# Autodesk Inventor assembly: robotassembly1
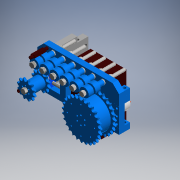
[picture p0: Inventor's stored thumbnail of the model, 180x180]
Saved by Autodesk Inventor 2016 (Build 200138000, 138)
## iProperties
Created: 2016-05-14
Part Number: robotassembly1
Document SubType Name: Assembly
Designer: hesaon
Author: hesaon
## Documents named in this file (22)
- C:\Users\hesaon\Documents\Killer-Bot-2016\AutodeskWorkspace\robotassembly1.iam
- C:\Users\hesaon\Documents\Killer-Bot-2016\AutodeskWorkspace\motorHolder57mmVer2.ipt
- C:\Users\hesaon\Documents\Killer-Bot-2016\AutodeskWorkspace\37D mm metal gearmotor.ipt
- C:\Users\hesaon\Documents\Killer-Bot-2016\AutodeskWorkspace\mountingHub6mm.ipt
- C:\Users\hesaon\Documents\Killer-Bot-2016\AutodeskWorkspace\sprocketsHolder.ipt
- C:\Users\hesaon\Documents\Killer-Bot-2016\AutodeskWorkspace\BigSprocket2.ipt
- C:\Users\hesaon\Documents\Killer-Bot-2016\AutodeskWorkspace\tracks_center.ipt
- C:\Users\hesaon\Documents\Killer-Bot-2016\AutodeskWorkspace\outerBigSprocket2.ipt
- C:\Users\hesaon\Documents\Killer-Bot-2016\AutodeskWorkspace\framesideRight.ipt
- C:\Users\hesaon\Documents\Killer-Bot-2016\AutodeskWorkspace\smallSprocketHolder.ipt
- C:\Users\hesaon\Documents\Killer-Bot-2016\AutodeskWorkspace\smallSprocket2.ipt
- C:\Users\hesaon\Documents\Killer-Bot-2016\AutodeskWorkspace\frameBack.ipt
- C:\Users\hesaon\Documents\Killer-Bot-2016\AutodeskWorkspace\pin5x60.ipt
- C:\Users\hesaon\Documents\Killer-Bot-2016\AutodeskWorkspace\smallSprocketFixture.ipt
- C:\Users\hesaon\Documents\Killer-Bot-2016\AutodeskWorkspace\roller.ipt
- C:\Users\hesaon\Documents\Killer-Bot-2016\AutodeskWorkspace\frameBottomRight.ipt
- C:\Users\hesaon\Documents\Killer-Bot-2016\AutodeskWorkspace\washer6mm.ipt
- C:\Users\hesaon\Documents\Killer-Bot-2016\AutodeskWorkspace\rollerdistance.ipt
- C:\Users\hesaon\Documents\Killer-Bot-2016\AutodeskWorkspace\nut6mm.ipt
- C:\Users\hesaon\Documents\Killer-Bot-2016\AutodeskWorkspace\bolt.ipt
- C:\Users\hesaon\Documents\Killer-Bot-2016\AutodeskWorkspace\battery.ipt
- C:\Users\hesaon\Documents\Killer-Bot-2016\AutodeskWorkspace\rollerdistanceShort.ipt
## Components (79 placed, 20 different names)
1. motorHolder57mmVer2:1 — Insert:1, Insert:2, Insert:98, Insert:99
2. 37D mm metal gearmotor:1 — Insert:1, Insert:2, Insert:3
3. mountingHub6mm:1 — Insert:3, Insert:9, Insert:10
4. sprocketsHolder:2 — Insert:7, Insert:8, Mate:1, Mate:2, Mate:3, Mate:4
5. Roller Chain Sprocket1:2 — Insert:7, Insert:8
6. Outer big sprocket:1 — Mate:1, Mate:2, Mate:3, Mate:4, Insert:9, Insert:10
7. framesideRight:1 — Flush:1, Insert:27, Insert:28, Insert:37, Flush:6, Flush:7, Insert:98, Insert:99, Insert:100, Insert:101, Mate:6, Mate:8
8. smallSprocketHolder:1 — Insert:13, Insert:14, Insert:15, Insert:16
9. Roller Chain Sprocket1:3 — Insert:13, Insert:14, Insert:93
10. Roller Chain Sprocket1:4 — Insert:15, Insert:16, Insert:17, Insert:92, Insert:94
11. tracks_center:2 — Insert:17
12. frameBack:1 — Flush:1, Flush:7, Insert:100, Insert:101
13. pin5x60:1 — Insert:27, Cylindrical:2
14. pin5x60:2 — Insert:28, Cylindrical:1
15. smallSprocketFixture:1 — Cylindrical:1, Cylindrical:2, Insert:91, Insert:95
16. roller:2 — Tangent:1, Flush:3, Flush:4, Insert:55, Insert:69, Insert:104
17. roller:3 — Insert:54, Insert:68, Insert:103, Insert:105
18. roller:4 — Insert:53, Insert:67, Insert:108
19. roller:5 — Insert:52, Insert:66, Insert:115
20. roller:6 — Insert:51, Insert:65, Insert:106
21. frameBottomRight:1 — Insert:37, Flush:6, Insert:71, Insert:72, Insert:73, Insert:74, Insert:75, Insert:76, Mate:7, Insert:103, Insert:104, Insert:105, Insert:106, Insert:107, Insert:108, Insert:115, Insert:116, Angle:1, Insert:117, Angle:2, Insert:118, Angle:3, Insert:119, Angle:4, Insert:120, Angle:5, Insert:121, Angle:6
22. tracks_center:3 — Tangent:1, Flush:3, Flush:4
23. roller:7 — Insert:50, Insert:64, Insert:107
24. washer6mm:1 — Insert:53, Insert:112
25. washer6mm:2 — Insert:51, Insert:110
26. washer6mm:3 — Insert:60
27. washer6mm:4 — Insert:59
28. washer6mm:5 — Insert:58
29. washer6mm:6 — Insert:61
30. washer6mm:7 — Insert:52, Insert:111
31. washer6mm:8 — Insert:56
32. washer6mm:9 — Insert:57
33. washer6mm:10 — Insert:55, Insert:114
34. washer6mm:11 — Insert:54, Insert:113
35. washer6mm:12 — Insert:50, Insert:109
36. rollerdistance:1 — Insert:61, Insert:114
37. rollerdistance:2 — Insert:59, Insert:112
38. rollerdistance:3 — Insert:60, Insert:113
39. rollerdistance:4 — Insert:58, Insert:111
40. rollerdistance:5 — Insert:57, Insert:110
41. rollerdistance:6 — Insert:56, Insert:109
42. nut6mm:1 — Insert:91, Insert:92, Insert:96
43. nut6mm:2 — Insert:90
44. nut6mm:3 — Insert:89
45. nut6mm:4 — Insert:88
46. nut6mm:5 — Insert:87
47. nut6mm:6 — Insert:86
48. nut6mm:7 — Insert:85
49. bolt:1 — Insert:80
50. bolt:2 — Insert:81
51. bolt:3 — Insert:82
52. bolt:4 — Insert:83
53. bolt:5 — Insert:97
54. bolt:6 — Insert:79
55. bolt:7 — Insert:78
56. washer6mm:13 — Insert:64, Insert:83
57. washer6mm:14 — Insert:65, Insert:82
58. washer6mm:15 — Insert:66, Insert:81
59. washer6mm:16 — Insert:67, Insert:80
60. washer6mm:17 — Insert:68, Insert:79
61. washer6mm:18 — Insert:69, Insert:78
62. washer6mm:19 — Insert:96, Insert:102
63. washer6mm:20 — Insert:93, Insert:97
64. washer6mm:21 — Insert:95
65. washer6mm:22 — Insert:94
66. washer6mm:23 — Insert:76, Insert:90
67. washer6mm:24 — Insert:72, Insert:86
68. washer6mm:25 — Insert:71, Insert:85
69. washer6mm:26 — Insert:75, Insert:89
70. washer6mm:27 — Insert:74, Insert:88
71. washer6mm:28 — Insert:73, Insert:87
72. battery:1 — Mate:6, Mate:7, Mate:8
73. rollerdistanceShort:1 — Insert:102
74. nut6mm:8 — Insert:116, Angle:1
75. nut6mm:9 — Insert:117, Angle:2
76. nut6mm:10 — Insert:118, Angle:3
77. nut6mm:11 — Insert:120, Angle:5
78. nut6mm:12 — Insert:121, Angle:6
79. nut6mm:13 — Insert:119, Angle:4
## Relationships (103: Insert 82, Mate 7, Angle 6, Flush 5, CylindricalJoint 2, Tangent 1)
- Insert:1: motorHolder57mmVer2:1 ↔ 37D mm metal gearmotor:1
- Insert:2: motorHolder57mmVer2:1 ↔ 37D mm metal gearmotor:1
- Insert:3: 37D mm metal gearmotor:1 ↔ mountingHub6mm:1
- Insert:7: sprocketsHolder:2 ↔ Roller Chain Sprocket1:2
- Insert:8: sprocketsHolder:2 ↔ Roller Chain Sprocket1:2
- Mate:1: sprocketsHolder:2 ↔ Outer big sprocket:1
- Mate:2: sprocketsHolder:2 ↔ Outer big sprocket:1
- Mate:3: sprocketsHolder:2 ↔ Outer big sprocket:1
- Mate:4: sprocketsHolder:2 ↔ Outer big sprocket:1
- Insert:9: mountingHub6mm:1 ↔ Outer big sprocket:1
- Insert:10: mountingHub6mm:1 ↔ Outer big sprocket:1
- Insert:13: smallSprocketHolder:1 ↔ Roller Chain Sprocket1:3
- Insert:14: smallSprocketHolder:1 ↔ Roller Chain Sprocket1:3
- Insert:15: smallSprocketHolder:1 ↔ Roller Chain Sprocket1:4
- Insert:16: smallSprocketHolder:1 ↔ Roller Chain Sprocket1:4
- Insert:17: Roller Chain Sprocket1:4 ↔ tracks_center:2
- Flush:1: framesideRight:1 ↔ frameBack:1
- Insert:27: framesideRight:1 ↔ pin5x60:1
- Insert:28: framesideRight:1 ↔ pin5x60:2
- Tangent:1: roller:2 ↔ tracks_center:3
- Flush:3: roller:2 ↔ tracks_center:3
- Flush:4: roller:2 ↔ tracks_center:3
- Insert:37: framesideRight:1 ↔ frameBottomRight:1
- Flush:6: framesideRight:1 ↔ frameBottomRight:1
- Insert:50: roller:7 ↔ washer6mm:12
- Insert:51: roller:6 ↔ washer6mm:2
- Insert:52: roller:5 ↔ washer6mm:7
- Insert:53: roller:4 ↔ washer6mm:1
- Insert:54: roller:3 ↔ washer6mm:11
- Insert:55: roller:2 ↔ washer6mm:10
- Insert:56: washer6mm:8 ↔ rollerdistance:6
- Insert:57: washer6mm:9 ↔ rollerdistance:5
- Insert:58: washer6mm:5 ↔ rollerdistance:4
- Insert:59: washer6mm:4 ↔ rollerdistance:2
- Insert:60: washer6mm:3 ↔ rollerdistance:3
- Insert:61: washer6mm:6 ↔ rollerdistance:1
- Flush:7: framesideRight:1 ↔ frameBack:1
- Insert:64: roller:7 ↔ washer6mm:13
- Insert:65: roller:6 ↔ washer6mm:14
- Insert:66: roller:5 ↔ washer6mm:15
- Insert:67: roller:4 ↔ washer6mm:16
- Insert:68: roller:3 ↔ washer6mm:17
- Insert:69: roller:2 ↔ washer6mm:18
- Insert:71: frameBottomRight:1 ↔ washer6mm:25
- Insert:72: frameBottomRight:1 ↔ washer6mm:24
- Insert:73: frameBottomRight:1 ↔ washer6mm:28
- Insert:74: frameBottomRight:1 ↔ washer6mm:27
- Insert:75: frameBottomRight:1 ↔ washer6mm:26
- Insert:76: frameBottomRight:1 ↔ washer6mm:23
- Insert:78: bolt:7 ↔ washer6mm:18
- Insert:79: bolt:6 ↔ washer6mm:17
- Insert:80: bolt:1 ↔ washer6mm:16
- Insert:81: bolt:2 ↔ washer6mm:15
- Insert:82: bolt:3 ↔ washer6mm:14
- Insert:83: bolt:4 ↔ washer6mm:13
- Insert:85: nut6mm:7 ↔ washer6mm:25
- Insert:86: nut6mm:6 ↔ washer6mm:24
- Insert:87: nut6mm:5 ↔ washer6mm:28
- Insert:88: nut6mm:4 ↔ washer6mm:27
- Insert:89: nut6mm:3 ↔ washer6mm:26
- Insert:90: nut6mm:2 ↔ washer6mm:23
- Cylindrical:1: pin5x60:2 ↔ smallSprocketFixture:1
- Cylindrical:2: pin5x60:1 ↔ smallSprocketFixture:1
- Insert:91: smallSprocketFixture:1 ↔ nut6mm:1
- Insert:92 (15 mm): Roller Chain Sprocket1:4 ↔ nut6mm:1
- Insert:93: Roller Chain Sprocket1:3 ↔ washer6mm:20
- Insert:94: Roller Chain Sprocket1:4 ↔ washer6mm:22
- Insert:95: smallSprocketFixture:1 ↔ washer6mm:21
- Insert:96: nut6mm:1 ↔ washer6mm:19
- Insert:97: bolt:5 ↔ washer6mm:20
- Insert:98: motorHolder57mmVer2:1 ↔ framesideRight:1
- Insert:99: motorHolder57mmVer2:1 ↔ framesideRight:1
- Insert:100: framesideRight:1 ↔ frameBack:1
- Insert:101: framesideRight:1 ↔ frameBack:1
- Insert:102: washer6mm:19 ↔ rollerdistanceShort:1
- Mate:6: framesideRight:1 ↔ battery:1
- Mate:7: frameBottomRight:1 ↔ battery:1
- Mate:8: framesideRight:1 ↔ battery:1
- Insert:103 (20.66 mm): roller:3 ↔ frameBottomRight:1
- Insert:104 (20.66 mm): roller:2 ↔ frameBottomRight:1
- Insert:105 (20.66 mm): roller:3 ↔ frameBottomRight:1
- Insert:106 (20.66 mm): roller:6 ↔ frameBottomRight:1
- Insert:107 (20.66 mm): frameBottomRight:1 ↔ roller:7
- Insert:108 (20.66 mm): roller:4 ↔ frameBottomRight:1
- Insert:109: washer6mm:12 ↔ rollerdistance:6
- Insert:110: washer6mm:2 ↔ rollerdistance:5
- Insert:111: washer6mm:7 ↔ rollerdistance:4
- Insert:112: washer6mm:1 ↔ rollerdistance:2
- Insert:113: washer6mm:11 ↔ rollerdistance:3
- Insert:114: washer6mm:10 ↔ rollerdistance:1
- Insert:115 (20.66 mm): roller:5 ↔ frameBottomRight:1
- Insert:116: frameBottomRight:1 ↔ nut6mm:8
- Angle:1 (0 deg): frameBottomRight:1 ↔ nut6mm:8
- Insert:117: frameBottomRight:1 ↔ nut6mm:9
- Angle:2 (0 deg): frameBottomRight:1 ↔ nut6mm:9
- Insert:118: frameBottomRight:1 ↔ nut6mm:10
- Angle:3 (0 deg): frameBottomRight:1 ↔ nut6mm:10
- Insert:119: frameBottomRight:1 ↔ nut6mm:13
- Angle:4 (0 deg): frameBottomRight:1 ↔ nut6mm:13
- Insert:120: frameBottomRight:1 ↔ nut6mm:11
- Angle:5 (0 deg): frameBottomRight:1 ↔ nut6mm:11
- Insert:121: frameBottomRight:1 ↔ nut6mm:12
- Angle:6 (0 deg): frameBottomRight:1 ↔ nut6mm:12
